# Autodesk Inventor assembly: s-assy-link4
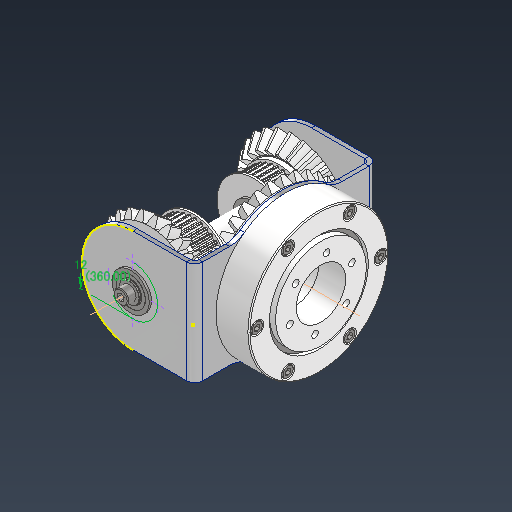
[picture p0: Inventor's stored thumbnail of the model, 512x512]
Saved by Autodesk Inventor 2021 (Build 250183000, 183)
## iProperties
Created: 2021-07-25
Part Number: s-assy-link4
Document SubType Name: Assembly
Designer: yuto6
Mass: 283.26 g
Surface Area: 777.393 cm^2
Volume: 130.987 cm^3
Density: 2.16251 g/cm^3
Author: yuto6
## Documents named in this file (15)
- C:\Users\yuta0\Desktop\cat_arm\s-assy-link4.iam
- C:\Users\yuta0\Desktop\cat_arm\s-assy-pulley-j4.iam
- C:\Users\yuta0\Desktop\cat_arm\alminium_plate1.ipt
- C:\Users\yuta0\Desktop\cat_arm\base10.ipt
- C:\Users\yuta0\Desktop\cat_arm\B6808ZZ.ipt
- C:\Users\yuta0\Desktop\cat_arm\base35.ipt
- C:\Users\yuta0\Desktop\cat_arm\FL688ZZ.ipt
- C:\Users\yuta0\Desktop\cat_arm\base7.ipt
- C:\Users\yuta0\Desktop\cat_arm\CB3-15.ipt
- C:\Users\yuta0\Desktop\cat_arm\base8.ipt
- C:\Users\yuta0\Desktop\cat_arm\base23.ipt
- C:\Users\yuta0\Desktop\cat_arm\SFHRW8-91-M4-N4.ipt
- C:\Users\yuta0\Desktop\cat_arm\CC-0814-05.ipt
- C:\Users\yuta0\Desktop\cat_arm\WSJ-STN-M4.ipt
- C:\Users\yuta0\Desktop\cat_arm\CB4-10.ipt
## Components (28 placed, 14 different names)
1. s-assy-pulley-j4:1 [sub-assembly] — メイト:15, メイト:20, メイト:25, メイト:26, メイト:38, メイト:41, メイト:47, メイト:51, メイト:52, メイト:53
2. alminium_plate1:1 — メイト:8, メイト:12, メイト:13, メイト:15, メイト:18, メイト:27, メイト:28, メイト:29, メイト:30
3. base10:1 — メイト:8, メイト:12, メイト:13, メイト:16, メイト:17, メイト:33, メイト:34
4. B6808ZZ:1 — メイト:16, メイト:18, メイト:19
5. B6808ZZ:2 — メイト:17, メイト:19, メイト:20, メイト:31, メイト:32
6. かさ歯車1:1 — メイト:22, メイト:24, メイト:25, メイト:26, メイト:39, メイト:44, メイト:55, メイト:56
7. FL688ZZ:1 — メイト:22, メイト:39, メイト:40
8. FL688ZZ:2 — メイト:24, メイト:40, メイト:58
9. FL688ZZ:3 — メイト:27, メイト:28, フラッシュ:1, メイト:57
10. FL688ZZ:4 — メイト:29, メイト:30, メイト:49, メイト:54
11. base7:1 — メイト:31, メイト:32, メイト:35, メイト:36, メイト:37, メイト:38
12. base8:1 — メイト:35, メイト:36, メイト:37
13. base23:1 — メイト:42, フラッシュ:2
14. SFHRW8-91-M4-N4:1 — メイト:41, メイト:42, フラッシュ:1, メイト:43, メイト:45
15. base34:1 — メイト:56, メイト:57
16. base34:2 — メイト:55, メイト:58
17. WSJ-STN-M4:1 — メイト:44, メイト:45, メイト:46
18. CB4-10:1 — メイト:43, メイト:46
19. CB4-10:2 — メイト:47, メイト:48, メイト:50
20. WSJ-STN-M4:2 — メイト:48, メイト:49, メイト:50
21. base34:3 — メイト:51, メイト:54
22. base34:4 — メイト:52, メイト:53
23. CB3-15:1 — メイト:33, メイト:34
24. CB3-15:2
25. CB3-15:3
26. CB3-15:4
27. CB3-15:5
28. CB3-15:6
## Component patterns: (6 elements, first: CB3-15:1)
## Relationships (47: Mate 45, Flush 2)
- メイト:8 [Mate]: alminium_plate1:1 ↔ base10:1
- メイト:12 [Mate]: alminium_plate1:1 ↔ base10:1
- メイト:13 [Mate]: alminium_plate1:1 ↔ base10:1
- メイト:15 [Mate]: s-assy-pulley-j4:1 ↔ alminium_plate1:1
- メイト:16 [Mate]: base10:1 ↔ B6808ZZ:1
- メイト:17 [Mate]: base10:1 ↔ B6808ZZ:2
- メイト:18 [Mate]: alminium_plate1:1 ↔ B6808ZZ:1
- メイト:19 [Mate]: B6808ZZ:1 ↔ B6808ZZ:2
- メイト:20 [Mate]: s-assy-pulley-j4:1 ↔ B6808ZZ:2
- メイト:22 [Mate]: かさ歯車1:1 ↔ FL688ZZ:1
- メイト:24 [Mate]: かさ歯車1:1 ↔ FL688ZZ:2
- メイト:25 [Mate]: s-assy-pulley-j4:1 ↔ かさ歯車1:1
- メイト:26 [Mate] (-36.395 mm): s-assy-pulley-j4:1 ↔ かさ歯車1:1
- メイト:27 [Mate]: alminium_plate1:1 ↔ FL688ZZ:3
- メイト:28 [Mate]: alminium_plate1:1 ↔ FL688ZZ:3
- メイト:29 [Mate]: alminium_plate1:1 ↔ FL688ZZ:4
- メイト:30 [Mate]: alminium_plate1:1 ↔ FL688ZZ:4
- メイト:31 [Mate]: B6808ZZ:2 ↔ base7:1
- メイト:32 [Mate]: B6808ZZ:2 ↔ base7:1
- メイト:33 [Mate]: base10:1 ↔ CB3-15:1
- メイト:34 [Mate]: base10:1 ↔ CB3-15:1
- メイト:35 [Mate]: base7:1 ↔ base8:1
- メイト:36 [Mate]: base7:1 ↔ base8:1
- メイト:37 [Mate]: base7:1 ↔ base8:1
- メイト:38 [Mate]: s-assy-pulley-j4:1 ↔ base7:1
- メイト:39 [Mate]: かさ歯車1:1 ↔ FL688ZZ:1
- メイト:40 [Mate]: FL688ZZ:1 ↔ FL688ZZ:2
- メイト:41 [Mate]: s-assy-pulley-j4:1 ↔ SFHRW8-91-M4-N4:1
- メイト:42 [Mate]: base23:1 ↔ SFHRW8-91-M4-N4:1
- フラッシュ:1 [Flush]: FL688ZZ:3 ↔ SFHRW8-91-M4-N4:1
- メイト:43 [Mate]: SFHRW8-91-M4-N4:1 ↔ CB4-10:1
- メイト:44 [Mate]: かさ歯車1:1 ↔ WSJ-STN-M4:1
- メイト:45 [Mate]: SFHRW8-91-M4-N4:1 ↔ WSJ-STN-M4:1
- メイト:46 [Mate]: WSJ-STN-M4:1 ↔ CB4-10:1
- メイト:47 [Mate]: s-assy-pulley-j4:1 ↔ CB4-10:2
- メイト:48 [Mate]: CB4-10:2 ↔ WSJ-STN-M4:2
- メイト:49 [Mate]: FL688ZZ:4 ↔ WSJ-STN-M4:2
- メイト:50 [Mate]: CB4-10:2 ↔ WSJ-STN-M4:2
- メイト:51 [Mate]: s-assy-pulley-j4:1 ↔ base34:3
- メイト:52 [Mate]: s-assy-pulley-j4:1 ↔ base34:4
- メイト:53 [Mate]: s-assy-pulley-j4:1 ↔ base34:4
- メイト:54 [Mate]: FL688ZZ:4 ↔ base34:3
- メイト:55 [Mate]: かさ歯車1:1 ↔ base34:2
- メイト:56 [Mate]: かさ歯車1:1 ↔ base34:1
- メイト:57 [Mate]: FL688ZZ:3 ↔ base34:1
- メイト:58 [Mate]: FL688ZZ:2 ↔ base34:2
- フラッシュ:2 [Flush]: base23:1
